# Autodesk Inventor assembly: Hatch design
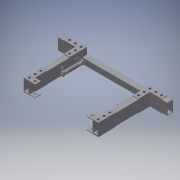
[picture p0: Inventor's stored thumbnail of the model, 180x180]
Saved by Autodesk Inventor 2018 (Build 220112000, 112)
## iProperties
Created: 2019-01-16
Part Number: Hatch design
Document SubType Name: Assembly
Designer: s-4008082
Author: s-4008082
## Documents named in this file (7)
- C:\Users\Burni\Desktop\Robotics\New Hatch\Hatch design.iam
- C:\Users\Burni\Desktop\Robotics\New Hatch\left arm.ipt
- C:\Users\Burni\Desktop\Robotics\New Hatch\right arm.ipt
- C:\Users\Burni\Desktop\Robotics\New Hatch\push bar.ipt
- C:\Users\Burni\Desktop\Robotics\New Hatch\PARTserver02019011803125824465437192d056f\AIS2018\021-DXP(F,D-770).iam
- C:\Users\Burni\Desktop\Robotics\New Hatch\bracing 2x3.ipt
- C:\Users\Burni\Desktop\Robotics\New Hatch\Bracing 3x3.ipt
## Components (13 placed, 6 different names)
1. left arm:1 — Mate:16, Flush:11, Mate:22, Mate:23, Flush:12, Flush:13, Mate:24, Flush:14, Flush:15, Flush:20, Flush:21, Mate:27, Mate:28, Flush:22, Flush:23, Flush:24, Mate:30, Flush:26
2. right arm:1 — Mate:17, Mate:18, Mate:19, Mate:20, Mate:21, Flush:16, Flush:17, Mate:25, Flush:18, Mate:26, Flush:19, Flush:24, Mate:30, Flush:25
3. push bar:1 — Mate:29, Mate:31, Mate:32, Mate:33
4. 021-DXP(F,D-770):1 [sub-assembly] — Mate:16, Mate:32, Mate:33, Flush:26
5. 021-DXP(F,D-770):2 [sub-assembly] — Mate:17, Mate:29, Mate:31, Flush:25
6. bracing 2x3:1 — Flush:11, Mate:22, Mate:23
7. bracing 2x3:2 — Flush:12, Flush:13, Mate:24, Flush:14, Flush:15
8. bracing 2x3:3 — Mate:20, Mate:21
9. bracing 2x3:4 — Mate:18, Mate:19
10. Bracing 3x3:1 — Flush:20, Flush:21, Mate:27
11. Bracing 3x3:2 — Mate:28, Flush:22, Flush:23
12. Bracing 3x3:3 — Flush:18, Mate:26, Flush:19
13. Bracing 3x3:4 — Flush:16, Flush:17, Mate:25
## Relationships (34: Mate 18, Flush 16)
- Mate:16: left arm:1 ↔ 021-DXP(F,D-770):1
- Mate:17: right arm:1 ↔ 021-DXP(F,D-770):2
- Mate:18: right arm:1 ↔ bracing 2x3:4
- Mate:19: right arm:1 ↔ bracing 2x3:4
- Mate:20: right arm:1 ↔ bracing 2x3:3
- Mate:21: right arm:1 ↔ bracing 2x3:3
- Flush:11: left arm:1 ↔ bracing 2x3:1
- Mate:22: left arm:1 ↔ bracing 2x3:1
- Mate:23: left arm:1 ↔ bracing 2x3:1
- Flush:12: left arm:1 ↔ bracing 2x3:2
- Flush:13: left arm:1 ↔ bracing 2x3:2
- Mate:24: left arm:1 ↔ bracing 2x3:2
- Flush:14: left arm:1 ↔ bracing 2x3:2
- Flush:15: left arm:1 ↔ bracing 2x3:2
- Flush:16: right arm:1 ↔ Bracing 3x3:4
- Flush:17: right arm:1 ↔ Bracing 3x3:4
- Mate:25: right arm:1 ↔ Bracing 3x3:4
- Flush:18: right arm:1 ↔ Bracing 3x3:3
- Mate:26: right arm:1 ↔ Bracing 3x3:3
- Flush:19: right arm:1 ↔ Bracing 3x3:3
- Flush:20: left arm:1 ↔ Bracing 3x3:1
- Flush:21: left arm:1 ↔ Bracing 3x3:1
- Mate:27: left arm:1 ↔ Bracing 3x3:1
- Mate:28: left arm:1 ↔ Bracing 3x3:2
- Flush:22: left arm:1 ↔ Bracing 3x3:2
- Flush:23: left arm:1 ↔ Bracing 3x3:2
- Flush:24: left arm:1 ↔ right arm:1
- Mate:29 (2.54 mm): push bar:1 ↔ 021-DXP(F,D-770):2
- Mate:30 (279.4 mm): left arm:1 ↔ right arm:1
- Mate:31: push bar:1 ↔ 021-DXP(F,D-770):2
- Mate:32 (2.54 mm): push bar:1 ↔ 021-DXP(F,D-770):1
- Mate:33: push bar:1 ↔ 021-DXP(F,D-770):1
- Flush:25 (38.1 mm): right arm:1 ↔ 021-DXP(F,D-770):2
- Flush:26 (38.1 mm): left arm:1 ↔ 021-DXP(F,D-770):1
